# Autodesk Inventor assembly: inner_mirrored
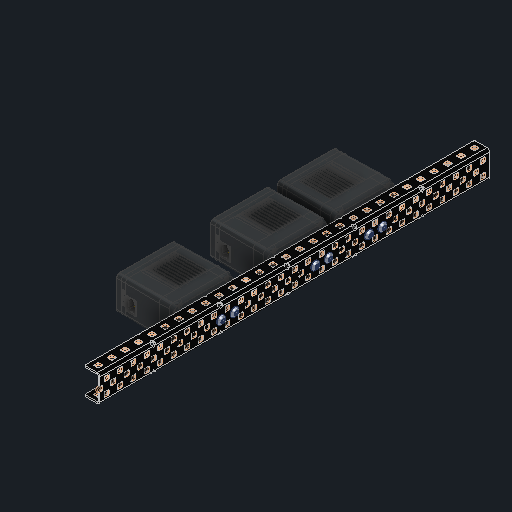
[picture p0: Inventor's stored thumbnail of the model, 512x512]
Saved by Autodesk Inventor 2024 (Build 280153000, 153)
## iProperties
Created: 2024-05-13
Part Number: inner_mirrored
Document SubType Name: Assembly
Designer: Averey Ku
Author: Averey Ku
## Documents named in this file (4)
- D:\vex_robotics\hardware\cad\kdot\chassis\drivebay\mirrored_parts\inner_mirrored.iam
- D:\vex_robotics\hardware\cad\kdot\chassis\drivebay\mirrored_parts\Alu C 1x2x1x29_mirrored.ipt
- D:\vex_robotics\hardware\cad\kdot\chassis\drivebay\mirrored_parts\.375 OD Aluminum Spacer 0.875_mirrored.ipt
- D:\vex_robotics\hardware\cad\kdot\chassis\drivebay\mirrored_parts\SteelM-StarS_mirrored.iam
## Components (6 placed, 3 different names)
1. Alu C 1x2x1x29_mirrored:1 — Insert:2, Insert:1, Mate:1, Insert:3, Insert:4, Mate:2, Insert:5
2. .375 OD Aluminum Spacer 0.875_mirrored:1 — Insert:2
3. .375 OD Aluminum Spacer 0.875_mirrored:2 — Insert:1
4. SteelM-StarS_mirrored:1 [sub-assembly] — Mate:1, Insert:3
5. SteelM-StarS_mirrored:2 [sub-assembly] — Insert:4
6. SteelM-StarS_mirrored:3 [sub-assembly] — Mate:2, Insert:5
## Relationships (7: Insert 5, Mate 2)
- Insert:2: Alu C 1x2x1x29_mirrored:1 ↔ .375 OD Aluminum Spacer 0.875_mirrored:1
- Insert:1: Alu C 1x2x1x29_mirrored:1 ↔ .375 OD Aluminum Spacer 0.875_mirrored:2
- Mate:1: Alu C 1x2x1x29_mirrored:1 ↔ SteelM-StarS_mirrored:1
- Insert:3: Alu C 1x2x1x29_mirrored:1 ↔ SteelM-StarS_mirrored:1
- Insert:4: Alu C 1x2x1x29_mirrored:1 ↔ SteelM-StarS_mirrored:2
- Mate:2: Alu C 1x2x1x29_mirrored:1 ↔ SteelM-StarS_mirrored:3
- Insert:5: Alu C 1x2x1x29_mirrored:1 ↔ SteelM-StarS_mirrored:3
